# Autodesk Inventor assembly: Linear Actuator
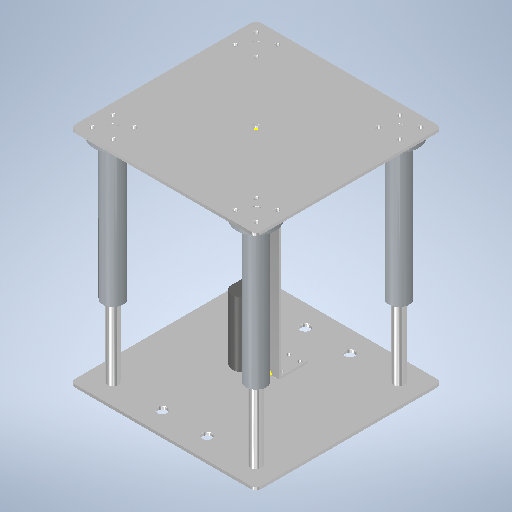
[picture p0: Inventor's stored thumbnail of the model, 512x512]
Saved by Autodesk Inventor 2025.3 (Build 293356000, 356)
## iProperties
Created: 2025-10-15
Part Number: Linear Actuator
Document SubType Name: Assembly
Designer: Haggag
Author: Haggag
## Documents named in this file (11)
- C:\Users\Haggag\Documents\Lifting Mechanism 150mm\Linear Actuator.iam
- C:\Users\Haggag\Documents\Lifting Mechanism 150mm\Actuonix-P16-150-256-12-P-Housing.ipt
- C:\Users\Haggag\Documents\Lifting Mechanism 150mm\Actuonix-P16-150-256-12-P-Shaft.ipt
- C:\Users\Haggag\Documents\Lifting Mechanism 150mm\Base.ipt
- C:\Users\Haggag\Documents\Lifting Mechanism 150mm\Linear Actuator Base Holder.ipt
- C:\Users\Haggag\Documents\Lifting Mechanism 150mm\Linear Actuator Plate Holder.ipt
- C:\Users\Haggag\Documents\Lifting Mechanism 150mm\Plate.ipt
- C:\Users\Haggag\Documents\Lifting Mechanism 150mm\Bracket Holder.ipt
- C:\Users\Haggag\Documents\Lifting Mechanism 150mm\Bracket.ipt
- C:\Users\Haggag\Documents\Lifting Mechanism 150mm\Plate Support.ipt
- C:\Users\Haggag\Documents\Lifting Mechanism 150mm\LMEF12LUU.ipt
## Components (16 placed, 10 different names)
1. Actuonix-P16-150-256-12-P-Housing:1 — Cylindrical:1, Rotational:2, Angle:1, Slider:1
2. Actuonix-P16-150-256-12-P-Shaft:1 — Cylindrical:1, Rigid:2
3. Base:2 — Rigid:1, Rigid:73, Rigid:74, Rigid:75, Rigid:76, Rigid:77
4. Linear Actuator Base Holder:1 — Rotational:2, Rigid:1
5. Linear Actuator Plate Holder:1 — Rigid:2, Rotational:5
6. Plate:1 — Rotational:5, Rigid:10, Rigid:13, Rigid:11, Rigid:12
7. Bracket Holder:1 — Rigid:3
8. Bracket:1 — Angle:1, Slider:1, Rigid:3
9. Plate Support:1 — Rigid:74, Rigid:77
10. Plate Support:2 — Rigid:73
11. Plate Support:3 — Rigid:75
12. Plate Support:4 — Rigid:76
13. LMEF12LUU:1 — Rigid:11
14. LMEF12LUU:2 — Rigid:12
15. LMEF12LUU:3 — Rigid:13
16. LMEF12LUU:4 — Rigid:10
## Relationships (17: WeldJoint 12, RevoluteJoint 2, CylindricalJoint 1, Angle 1, TranslationJoint 1)
- Cylindrical:1: Actuonix-P16-150-256-12-P-Housing:1 ↔ Actuonix-P16-150-256-12-P-Shaft:1
- Rotational:2 [RevoluteJoint]: Actuonix-P16-150-256-12-P-Housing:1 ↔ Linear Actuator Base Holder:1
- Rigid:1 [WeldJoint]: Base:2 ↔ Linear Actuator Base Holder:1
- Rigid:2 [WeldJoint] (-0.7 mm): Actuonix-P16-150-256-12-P-Shaft:1 ↔ Linear Actuator Plate Holder:1
- Rotational:5 [RevoluteJoint]: Linear Actuator Plate Holder:1 ↔ Plate:1
- Angle:1 (0 deg): Actuonix-P16-150-256-12-P-Housing:1 ↔ Bracket:1
- Slider:1 [TranslationJoint]: Actuonix-P16-150-256-12-P-Housing:1 ↔ Bracket:1
- Rigid:3 [WeldJoint]: Bracket Holder:1 ↔ Bracket:1
- Rigid:10 [WeldJoint]: Plate:1 ↔ LMEF12LUU:4
- Rigid:13 [WeldJoint]: Plate:1 ↔ LMEF12LUU:3
- Rigid:11 [WeldJoint]: Plate:1 ↔ LMEF12LUU:1
- Rigid:12 [WeldJoint]: Plate:1 ↔ LMEF12LUU:2
- Rigid:73 [WeldJoint]: Base:2 ↔ Plate Support:2
- Rigid:74 [WeldJoint]: Base:2 ↔ Plate Support:1
- Rigid:75 [WeldJoint]: Base:2 ↔ Plate Support:3
- Rigid:76 [WeldJoint]: Base:2 ↔ Plate Support:4
- Rigid:77 [WeldJoint]: Base:2 ↔ Plate Support:1
